# Autodesk Inventor assembly: 210-110c
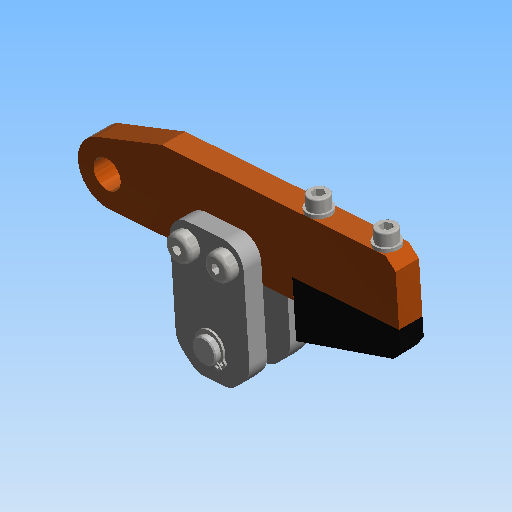
[picture p0: Inventor's stored thumbnail of the model, 512x512]
Saved by Autodesk Inventor 2020.1 (Build 241239000, 239)
## iProperties
Created: 2006-02-01
Part Number: 210-110c
Document SubType Name: Assembly
Designer: Kevin
Manufacturer: Standard
Standards Organization: Custom
Description: CLAMP UNIT FRONT FINGER
Weld Material: Default
Title: ASSEMBLY
Author: Kevin
Revision Number: -
## Documents named in this file (11)
- C:\Users\thom_tremblay\Desktop\Inventor ACP Data\Assemblies\210-110c.IAM
- C:\Users\thom_tremblay\Desktop\Inventor ACP Data\Parts\210-106c.ipt
- C:\Users\thom_tremblay\Desktop\Inventor ACP Data\Parts\210-107c.ipt
- C:\Users\thom_tremblay\Desktop\Inventor ACP Data\Parts\210-108c.ipt
- C:\Users\thom_tremblay\Desktop\Inventor ACP Data\Parts\210-109c.ipt
- C:\Users\thom_tremblay\Desktop\Inventor ACP Data\Content Center\en-US\ISO 7379\8-30.ipt
- C:\Users\thom_tremblay\Desktop\Inventor ACP Data\Content Center\en-US\ISO 7089\8.ipt
- C:\Users\thom_tremblay\Desktop\Inventor ACP Data\Content Center\en-US\ISO 4032\M6.ipt
- C:\Users\thom_tremblay\Desktop\Inventor ACP Data\Content Center\en-US\DIN 471  _ 9mm _= 300mm\12-11.5-1.ipt
- C:\Users\thom_tremblay\Desktop\Inventor ACP Data\Content Center\en-US\ISO 4762\M6-45.ipt
- C:\Users\thom_tremblay\Desktop\Inventor ACP Data\Content Center\en-US\ISO 7089\6.ipt
## Components (17 placed, 10 different names)
1. 210-106c:1 — Mate:10
2. 210-107c:1 — Mate:10, Mate:11, Insert:3, Insert:4
3. 210-108c:1
4. 210-109c:1 — Mate:7, Mate:8, Mate:9, Mate:11, Insert:9, Insert:10
5. 210-106c:2 — Mate:7, Mate:8, Mate:9, Insert:1, Insert:2
6. "ISO 7379 " 8  x 30:1 — Insert:1, Insert:5
7. "ISO 7089" 8 - 140 HV:1 — Insert:6, Insert:8
8. "ISO 7089" 8 - 140 HV:2 — Insert:5, Insert:7
9. "ISO 4032 " M6:1 — Insert:7
10. "ISO 7379 " 8  x 30:2 — Insert:2, Insert:6
11. "ISO 4032 " M6:2 — Insert:8
12. "DIN 471  > 9mm <= 300mm" 12 x 1:1 — Insert:4
13. "DIN 471  > 9mm <= 300mm" 12 x 1:2 — Insert:3
14. "ISO 4762 " M6 x 45:1 — Insert:11
15. "ISO 7089" 6 - 140 HV:1 — Insert:10, Insert:11
16. "ISO 4762 " M6 x 45:2 — Insert:12
17. "ISO 7089" 6 - 140 HV:2 — Insert:9, Insert:12
## Relationships (23: Insert 12, Mate 11)
- [Mate]: 210-106c:1 ↔ 210-109c:1
- [Mate]: 210-106c:1 ↔ 210-109c:1
- [Mate]: 210-106c:1 ↔ 210-109c:1
- [Mate]: 210-108c:1 ↔ 210-109c:1
- [Mate]: 210-108c:1 ↔ 210-109c:1
- [Mate]: 210-108c:1 ↔ 210-109c:1
- Mate:7: 210-109c:1 ↔ 210-106c:2
- Mate:8: 210-109c:1 ↔ 210-106c:2
- Mate:9: 210-109c:1 ↔ 210-106c:2
- Mate:10: 210-106c:1 ↔ 210-107c:1
- Mate:11: 210-107c:1 ↔ 210-109c:1
- Insert:1: 210-106c:2 ↔ "ISO 7379 " 8  x 30:1
- Insert:2: 210-106c:2 ↔ "ISO 7379 " 8  x 30:2
- Insert:3: 210-107c:1 ↔ "DIN 471  > 9mm <= 300mm" 12 x 1:2
- Insert:4: 210-107c:1 ↔ "DIN 471  > 9mm <= 300mm" 12 x 1:1
- Insert:5: "ISO 7379 " 8  x 30:1 ↔ "ISO 7089" 8 - 140 HV:2
- Insert:6: "ISO 7089" 8 - 140 HV:1 ↔ "ISO 7379 " 8  x 30:2
- Insert:7: "ISO 7089" 8 - 140 HV:2 ↔ "ISO 4032 " M6:1
- Insert:8: "ISO 7089" 8 - 140 HV:1 ↔ "ISO 4032 " M6:2
- Insert:9: 210-109c:1 ↔ "ISO 7089" 6 - 140 HV:2
- Insert:10: 210-109c:1 ↔ "ISO 7089" 6 - 140 HV:1
- Insert:11: "ISO 4762 " M6 x 45:1 ↔ "ISO 7089" 6 - 140 HV:1
- Insert:12: "ISO 4762 " M6 x 45:2 ↔ "ISO 7089" 6 - 140 HV:2
